# Autodesk Inventor assembly: belt reduction
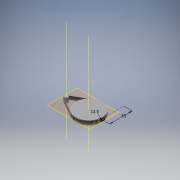
[picture p0: Inventor's stored thumbnail of the model, 180x180]
Saved by Autodesk Inventor 2017 (Build 210142000, 142)
## iProperties
Created: 2018-04-16
Part Number: belt reduction
Document SubType Name: Assembly
Designer: RKL
Author: RKL
## Documents named in this file (3)
- E:\st motor\rotary die grinder engine\transmission\belt reduction\belt reduction.iam
- E:\st motor\rotary die grinder engine\transmission\belt reduction\belt reduction\Design Accelerator\Synchronous Belts Transmission1.iam
- E:\st motor\rotary die grinder engine\transmission\belt reduction\baseplate.ipt
## Components (2 placed, 2 different names)
1. Synchronous Belts Transmission:1 [sub-assembly]
2. baseplate:1 — Flush:1, Flush:2
## Relationships (2: Flush 2)
- Flush:1: baseplate:1
- Flush:2: baseplate:1
